# Autodesk Inventor assembly: ThunderhexPostWithBearing
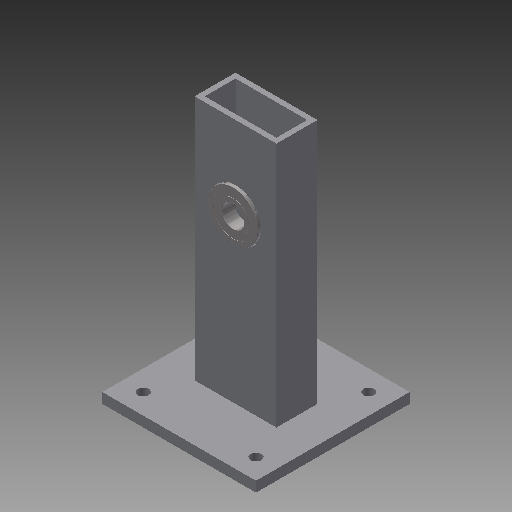
[picture p0: Inventor's stored thumbnail of the model, 512x512]
Saved by Autodesk Inventor 2017 SP1 (Build 210196100, 196)
## iProperties
Created: 2016-08-08
Part Number: ThunderhexPostWithBearing
Document SubType Name: Assembly
Designer: steele
Author: steele
## Documents named in this file (3)
- D:\snobotics\CAD-Development\robSteele\SnoBotics2016\2016-08-05-TiltWithVex\ThunderhexPostWithBearing.iam
- D:\snobotics\CAD-Development\robSteele\SnoBotics2016\2016-08-05-TiltWithVex\ThunderhexPost.ipt
- D:\snobotics\CAD-MfgResources\VexRobotics\ThunderHex\217-4006-STEP-20140807.ipt
## Components (2 placed, 2 different names)
1. ThunderhexPost:1 — Insert:1
2. 217-4006-STEP-20140807:1 — Insert:1
## Relationships (1: Insert 1)
- Insert:1: ThunderhexPost:1 ↔ 217-4006-STEP-20140807:1
